# Autodesk Inventor assembly: Relaismodul Baugruppe
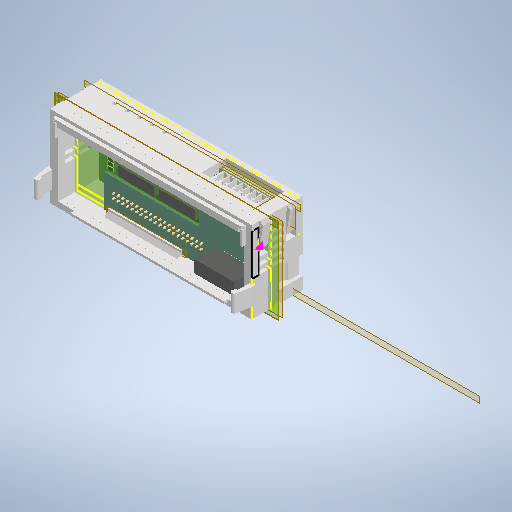
[picture p0: Inventor's stored thumbnail of the model, 512x512]
Saved by Autodesk Inventor 2025.2 (Build 292293000, 293)
## iProperties
Created: 2025-11-05
Part Number: Relaismodul Baugruppe
Document SubType Name: Assembly
Designer: leowa
Author: leowa
## Documents named in this file (4)
- C:\Users\leowa\OneDrive - Fachhochschule Aachen\FH\8. Semester\CAN Tram CAD\Module\Relaismodul Baugruppe.iam
- C:\Users\leowa\OneDrive - Fachhochschule Aachen\FH\8. Semester\CAN Tram CAD\Gehäuse\Relais Gehäuse.ipt
- C:\Users\leowa\OneDrive - Fachhochschule Aachen\FH\8. Semester\CAN Tram CAD\Platinen\Relaismodul\Relaismodul\Relaismodul.iam
- C:\Users\leowa\OneDrive - Fachhochschule Aachen\FH\8. Semester\CAN Tram CAD\Gehäuse\Relais Gehäuse Deckel.ipt
## Components (3 placed, 3 different names)
1. Relais Gehäuse:1 — Passend:1, Passend:2, Passend:3, Fluchtend:1, Fluchtend:2, Passend:4
2. Relaismodul:1 [sub-assembly] — Passend:1, Passend:2, Passend:3
3. Relais Gehäuse Deckel:1 — Fluchtend:1, Fluchtend:2, Passend:4
## Relationships (6: Mate 4, Flush 2)
- Passend:1 [Mate]: Relais Gehäuse:1 ↔ Relaismodul:1
- Passend:2 [Mate] (1 mm): Relais Gehäuse:1 ↔ Relaismodul:1
- Passend:3 [Mate]: Relais Gehäuse:1 ↔ Relaismodul:1
- Fluchtend:1 [Flush]: Relais Gehäuse:1 ↔ Relais Gehäuse Deckel:1
- Fluchtend:2 [Flush]: Relais Gehäuse:1 ↔ Relais Gehäuse Deckel:1
- Passend:4 [Mate]: Relais Gehäuse:1 ↔ Relais Gehäuse Deckel:1
